# Autodesk Inventor assembly: octoBotoAssembly01
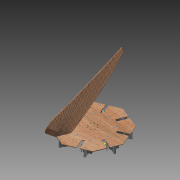
[picture p0: Inventor's stored thumbnail of the model, 180x180]
Saved by Autodesk Inventor 2013 (Build 170138000, 138)
## iProperties
Created: 2014-08-20
Part Number: octoBotoAssembly01
Document SubType Name: Assembly
Designer: Nano
Author: Nano
## Documents named in this file (5)
- C:\Users\Nano\Documents\InventorByron\InventorMasterProject\octoBoto\octoBotoAssembly01.iam
- C:\Users\Nano\Documents\InventorByron\InventorMasterProject\octoBoto\octoBoto01.ipt
- C:\Users\Nano\Documents\InventorByron\InventorMasterProject\octoBoto\HS-311 Hitec Standard Servo and Horn.iam
- C:\Users\Nano\Documents\InventorByron\InventorMasterProject\octoBoto\servoMountPlate.ipt
- C:\Users\Nano\Documents\InventorByron\InventorMasterProject\octoBoto\octoBotoWing01.ipt
## Components (18 placed, 4 different names)
1. octoBoto01:1 — Mate:1, Flush:1, Mate:2, Flush:2, Flush:3
2. octoBotoWing01:1 — Mate:3, Mate:4
3. servoMountPlate:1 — Flush:2, Flush:3
4. servoMountPlate:2
5. servoMountPlate:3
6. servoMountPlate:4
7. servoMountPlate:5
8. servoMountPlate:6
9. servoMountPlate:7
10. servoMountPlate:8
11. HS-311 Hitec Standard Servo and Horn:1 [sub-assembly] — Mate:1, Flush:1, Mate:2, Mate:3, Mate:4
12. HS-311 Hitec Standard Servo and Horn:2 [sub-assembly]
13. HS-311 Hitec Standard Servo and Horn:3 [sub-assembly]
14. HS-311 Hitec Standard Servo and Horn:4 [sub-assembly]
15. HS-311 Hitec Standard Servo and Horn:5 [sub-assembly]
16. HS-311 Hitec Standard Servo and Horn:6 [sub-assembly]
17. HS-311 Hitec Standard Servo and Horn:7 [sub-assembly]
18. HS-311 Hitec Standard Servo and Horn:8 [sub-assembly]
## Component patterns: (8 elements, first: servoMountPlate:1), (8 elements, first: HS-311 Hitec Standard Servo and Horn:1)
## Relationships (7: Mate 4, Flush 3)
- Mate:1: octoBoto01:1 ↔ HS-311 Hitec Standard Servo and Horn:1
- Flush:1 (-12.7 mm): octoBoto01:1 ↔ HS-311 Hitec Standard Servo and Horn:1
- Mate:2 (1.5875 mm): octoBoto01:1 ↔ HS-311 Hitec Standard Servo and Horn:1
- Flush:2: octoBoto01:1 ↔ servoMountPlate:1
- Flush:3: octoBoto01:1 ↔ servoMountPlate:1
- Mate:3: octoBotoWing01:1 ↔ HS-311 Hitec Standard Servo and Horn:1
- Mate:4: octoBotoWing01:1 ↔ HS-311 Hitec Standard Servo and Horn:1
